# Autodesk Inventor assembly: CameraUnit
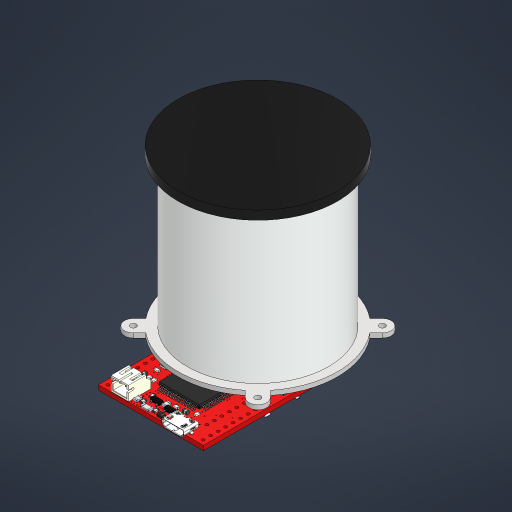
[picture p0: Inventor's stored thumbnail of the model, 512x512]
Saved by Autodesk Inventor 2024.2 (Build 282272000, 272)
## iProperties
Created: 2023-12-21
Part Number: CameraUnit
Document SubType Name: Assembly
Designer: Hanaoka
Author: Hanaoka
## Documents named in this file (5)
- G:\共有ドライブ\reRo\05_個人\hanaoka\inventor\CameraUnit\CameraUnit.iam
- G:\共有ドライブ\reRo\05_個人\hanaoka\inventor\CameraUnit\Camera_pipe.ipt
- G:\共有ドライブ\reRo\05_個人\hanaoka\inventor\CameraUnit\Camera_mirror.ipt
- G:\共有ドライブ\reRo\05_個人\hanaoka\inventor\CameraUnit\OpenMV_H7\OpenMV_H7.iam
- G:\共有ドライブ\reRo\05_個人\hanaoka\inventor\CameraUnit\Camera_Mount.ipt
## Components (4 placed, 4 different names)
1. Camera_pipe:1 — 挿入:1, 挿入:2
2. Camera_mirror:1 — 挿入:2
3. OpenMV_H7:1 [sub-assembly] — メイト:1, フラッシュ:1, メイト:2, フラッシュ:2
4. Camera_Mount:1 — フラッシュ:2, 挿入:1
## Relationships (6: Mate 2, Flush 2, Insert 2)
- メイト:1 [Mate]: OpenMV_H7:1
- フラッシュ:1 [Flush]: OpenMV_H7:1
- メイト:2 [Mate]: OpenMV_H7:1
- フラッシュ:2 [Flush]: OpenMV_H7:1 ↔ Camera_Mount:1
- 挿入:1 [Insert]: Camera_pipe:1 ↔ Camera_Mount:1
- 挿入:2 [Insert]: Camera_pipe:1 ↔ Camera_mirror:1
